# Autodesk Inventor assembly: 28_Horn_Set
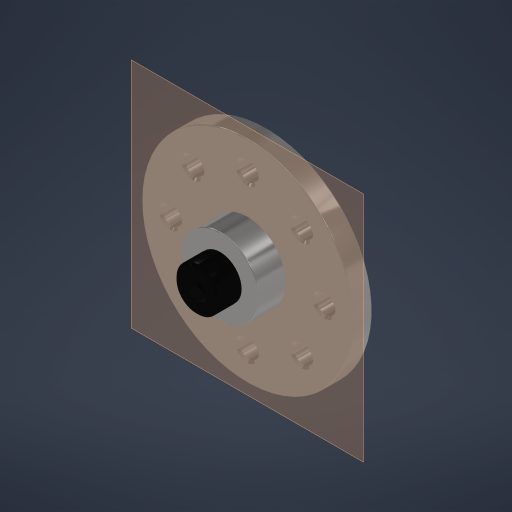
[picture p0: Inventor's stored thumbnail of the model, 512x512]
Saved by Autodesk Inventor 2024 (Build 280153000, 153)
## iProperties
Created: 2024-02-15
Part Number: 28_Horn_Set
Document SubType Name: Assembly
Designer: ASUS
Author: ASUS
## Documents named in this file (3)
- C:\Users\ASUS\Desktop\Anti_Backlash_Structure_OP\ROBOTIS(Inventor 2024 ver.)\혼\28_Horn_Set.iam
- C:\Users\ASUS\Desktop\Anti_Backlash_Structure_OP\ROBOTIS(Inventor 2024 ver.)\혼\28Horn.ipt
- C:\Users\ASUS\Desktop\Anti_Backlash_Structure_OP\MISUMI\CSH-ST-M2_5-10_203.ipt
## Components (2 placed, 2 different names)
1. 28Horn:2 — 삽입:1
2. CSH-ST-M2_5-10_203:1 — 삽입:1
## Relationships (1: Insert 1)
- 삽입:1 [Insert]: 28Horn:2 ↔ CSH-ST-M2_5-10_203:1
